# Autodesk Inventor assembly: 組合
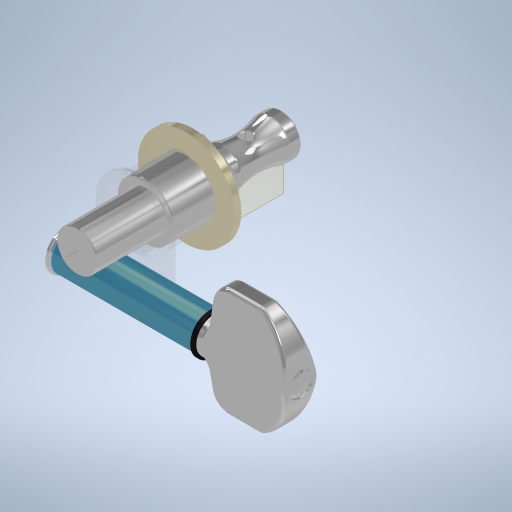
[picture p0: Inventor's stored thumbnail of the model, 512x512]
Saved by Autodesk Inventor 2024.2 (Build 282272000, 272)
## iProperties
Created: 2024-05-09
Part Number: 組合
Document SubType Name: Assembly
Designer: User
Author: User
## Documents named in this file (12)
- C:\Users\User\OneDrive - 國立中山大學\桌面\創客基礎\0509\組合.iam
- C:\Users\User\Downloads\零件附件檔\CH5-Assembly 1\CH5-Assembly 1\casting2.ipt
- C:\Users\User\Downloads\零件附件檔\CH5-Assembly 1\CH5-Assembly 1\large cap.ipt
- C:\Users\User\Downloads\零件附件檔\CH5-Assembly 1\CH5-Assembly 1\small cap.ipt
- C:\Users\User\Downloads\零件附件檔\CH5-Assembly 1\CH5-Assembly 1\shaft.ipt
- C:\Users\User\Downloads\零件附件檔\CH5-Assembly 1\CH5-Assembly 1\thrust washer.ipt
- C:\Users\User\Downloads\零件附件檔\CH5-Assembly 1\CH5-Assembly 1\button.ipt
- C:\Users\User\Downloads\零件附件檔\CH5-Assembly 1\CH5-Assembly 1\screw.ipt
- C:\Users\User\Downloads\零件附件檔\CH5-Assembly 1\CH5-Assembly 1\postcap.ipt
- C:\Users\User\Downloads\零件附件檔\CH5-Assembly 1\CH5-Assembly 1\trim washer.ipt
- C:\Users\User\Downloads\零件附件檔\CH5-Assembly 1\CH5-Assembly 1\hex sleeve.ipt
- C:\Users\User\Downloads\零件附件檔\CH5-Assembly 1\CH5-Assembly 1\string post.ipt
## Components (11 placed, 11 different names)
1. casting2:1 — 齊平:1, 貼合:1, 齊平:2, 貼合:2, 貼合:3, 貼合:4, 貼合:8, 角度:1, 貼合:9, 貼合:10, 貼合:11, 貼合:17
2. large cap:1 — 齊平:1, 貼合:1, 貼合:16
3. small cap:1 — 齊平:2, 貼合:2
4. shaft:1 — 貼合:3, 貼合:4, 貼合:5, 貼合:6, 插入:1
5. thrust washer:1 — 貼合:5, 貼合:6, 貼合:7
6. button:1 — 貼合:7, 貼合:8, 角度:1
7. screw:1 — 插入:1
8. postcap:1 — 貼合:9, 貼合:10, 貼合:11, 貼合:12, 貼合:13, 貼合:15
9. trim washer:1 — 貼合:12, 貼合:13, 貼合:14
10. hex sleeve:1 — 貼合:14, 貼合:15
11. string post:1 — 貼合:16, 貼合:17, 貼合:18, 貼合:19
## Relationships (25: Mate 21, Flush 2, Angle 1, Insert 1)
- 齊平:1 [Flush]: casting2:1 ↔ large cap:1
- 貼合:1 [Mate]: casting2:1 ↔ large cap:1
- 齊平:2 [Flush]: casting2:1 ↔ small cap:1
- 貼合:2 [Mate]: casting2:1 ↔ small cap:1
- 貼合:3 [Mate]: casting2:1 ↔ shaft:1
- 貼合:4 [Mate]: casting2:1 ↔ shaft:1
- 貼合:5 [Mate]: shaft:1 ↔ thrust washer:1
- 貼合:6 [Mate]: shaft:1 ↔ thrust washer:1
- 貼合:7 [Mate]: thrust washer:1 ↔ button:1
- 貼合:8 [Mate]: casting2:1 ↔ button:1
- 角度:1 [Angle] (10 deg): casting2:1 ↔ button:1
- 插入:1 [Insert]: shaft:1 ↔ screw:1
- 貼合:9 [Mate]: casting2:1 ↔ postcap:1
- 貼合:10 [Mate]: casting2:1 ↔ postcap:1
- 貼合:11 [Mate]: casting2:1 ↔ postcap:1
- 貼合:12 [Mate]: postcap:1 ↔ trim washer:1
- 貼合:13 [Mate]: postcap:1 ↔ trim washer:1
- 貼合:14 [Mate]: trim washer:1 ↔ hex sleeve:1
- 貼合:15 [Mate]: postcap:1 ↔ hex sleeve:1
- 貼合:16 [Mate]: large cap:1 ↔ string post:1
- 貼合:17 [Mate]: casting2:1 ↔ string post:1
- 貼合:18 [Mate]: string post:1
- 貼合:19 [Mate]: string post:1
- 貼合:20 [Mate]
- 貼合:21 [Mate]
